# Autodesk Inventor assembly: ServoAndHorn
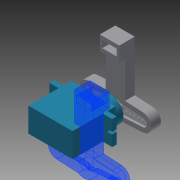
[picture p0: Inventor's stored thumbnail of the model, 180x180]
Saved by Autodesk Inventor 2014 SP1 (Build 180222100, 222)
## iProperties
Created: 2017-05-14
Part Number: ServoAndHorn
Document SubType Name: Assembly
Designer: danielsikar
Author: danielsikar
## Documents named in this file (4)
- C:\Users\danielsikar\Documents\Inventor\FlaskCradle\assemblies\ServoAndHorn.iam
- C:\Users\danielsikar\Documents\Inventor\FlaskCradle\parts\Servo.ipt
- C:\Users\danielsikar\Documents\Inventor\FlaskCradle\parts\ServoBlade.ipt
- C:\Users\danielsikar\Documents\Inventor\FlaskCradle\parts\HornPocket.ipt
## Components (3 placed, 3 different names)
1. Servo:1 — Mate:1, Mate:2, Mate:3, Mate:4
2. ServoBlade:1 — Mate:3, Mate:4, Mate:5, Flush:2
3. HornPocket:1 — Flush:1, Flush:2
## Relationships (7: Mate 5, Flush 2)
- Mate:1: Servo:1
- Mate:2: Servo:1
- Mate:3: Servo:1 ↔ ServoBlade:1
- Mate:4: Servo:1 ↔ ServoBlade:1
- Mate:5 (6.25 mm): ServoBlade:1
- Flush:1: HornPocket:1
- Flush:2: ServoBlade:1 ↔ HornPocket:1
